# Autodesk Inventor assembly: gear_hub
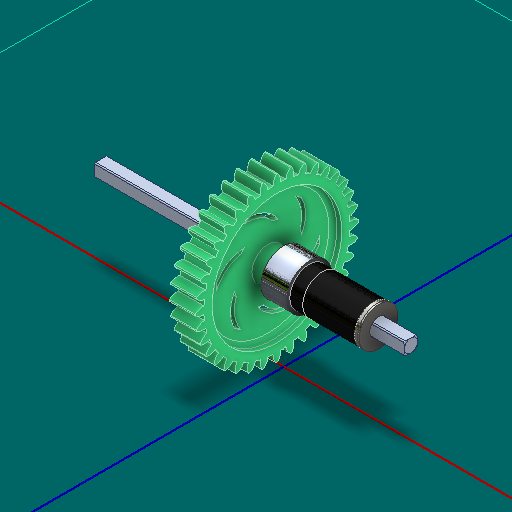
[picture p0: Inventor's stored thumbnail of the model, 512x512]
Saved by Autodesk Inventor 2025 (Build 290162000, 162)
## iProperties
Created: 2024-08-23
Part Number: gear_hub
Document SubType Name: Assembly
Designer: averey
Author: averey
## Documents named in this file (12)
- C:\Users\avere\vex_robotics_high_stakes\hardware\cad\bots\CRAY-1\chassis\drivetrain\drivebay\gear_hub.iam
- C:\Users\avere\vex_robotics_high_stakes\hardware\cad\VEX-CAD-Inventor\Motion\Gears\LS 36T Gear.ipt
- C:\Users\avere\vex_robotics_high_stakes\hardware\cad\VEX-CAD-Inventor\Motion\Spacers\Spacer Nylon .375 OD\NSpacer .375 OD x .125.ipt
- C:\Users\avere\vex_robotics_high_stakes\hardware\cad\VEX-CAD-Inventor\Motion\Spacers\Spacer Nylon .375 OD.ipt
- C:\Users\avere\vex_robotics_high_stakes\hardware\cad\VEX-CAD-Inventor\Motion\Spacers\Spacer Nylon .375 OD\NSpacer .375 OD x .500.ipt
- C:\Users\avere\vex_robotics_high_stakes\hardware\cad\VEX-CAD-Inventor\Motion\Shaft LS\Shaft Collar ipts\Shaft Collar Set Screw.ipt
- C:\Users\avere\vex_robotics_high_stakes\hardware\cad\VEX-CAD-Inventor\Motion\Spacers\Washer Steel\SWasher .375 OD x .031250.ipt
- C:\Users\avere\vex_robotics_high_stakes\hardware\cad\VEX-CAD-Inventor\Motion\Spacers\Washer Steel.ipt
- C:\Users\avere\vex_robotics_high_stakes\hardware\cad\VEX-CAD-Inventor\Motion\Spacers\Washer Steel\SWasher .375 OD x .015625.ipt
- C:\Users\avere\vex_robotics_high_stakes\hardware\cad\VEX-CAD-Inventor\Motion\Spacers\Washer Steel\SWasher .375 OD x .062500.ipt
- C:\Users\avere\vex_robotics_high_stakes\hardware\cad\VEX-CAD-Inventor\Motion\Shaft LS\Shaft LS\Shaft LS 3.0.ipt
- C:\Users\avere\vex_robotics_high_stakes\hardware\cad\VEX-CAD-Inventor\Motion\Shaft LS\Shaft LS.ipt
## Components (8 placed, 8 different names)
1. LS 36T Gear:1
2. NSpacer .375 OD x .125:1
3. NSpacer .375 OD x .500:2
4. Shaft Collar Set Screw:1 — Mate:1
5. SWasher .375 OD x .031250:1
6. SWasher .375 OD x .015625:2 — Insert:7
7. SWasher .375 OD x .062500:3
8. Shaft LS 3.0:1 — Insert:7
## Relationships (8: Insert 7, Mate 1)
- [Insert]: NSpacer .375 OD x .125:1 ↔ NSpacer .375 OD x .500:2
- [Insert]: NSpacer .375 OD x .125:1 ↔ Shaft Collar Set Screw:1
- [Insert]: SWasher .375 OD x .031250:1 ↔ SWasher .375 OD x .015625:2
- [Insert]: NSpacer .375 OD x .500:2 ↔ SWasher .375 OD x .031250:1
- [Insert]: LS 36T Gear:1 ↔ Shaft Collar Set Screw:1
- [Insert]: LS 36T Gear:1 ↔ SWasher .375 OD x .062500:3
- Mate:1: Shaft Collar Set Screw:1
- Insert:7 (-7.9375 mm): SWasher .375 OD x .015625:2 ↔ Shaft LS 3.0:1
